# Autodesk Inventor assembly: 4x2
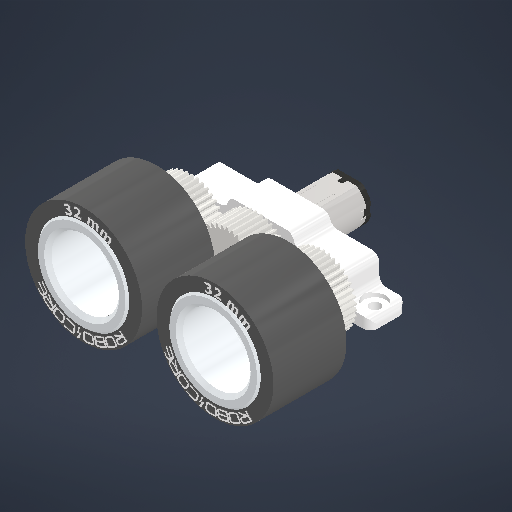
[picture p0: Inventor's stored thumbnail of the model, 512x512]
Saved by Autodesk Inventor 2026.1 (Build 301233020, 233B)
## iProperties
Created: 2026-02-10
Part Number: 4x2
Document SubType Name: Assembly
Designer: celio
Author: celio
## Documents named in this file (6)
- C:\Users\celio\OneDrive\Documentos\Inventor\ZeGuia\Montagem\4x2\Base\4x2.iam
- C:\Users\celio\OneDrive\Documentos\Inventor\ZeGuia\Roda\Roda.iam
- C:\Users\celio\OneDrive\Documentos\Inventor\ZeGuia\Motores\N20\N20 DC MOTOR.ipt
- C:\Users\celio\OneDrive\Documentos\Inventor\ZeGuia\Montagem\4x2\Suporte.ipt
- C:\Users\celio\OneDrive\Documentos\Inventor\ZeGuia\Montagem\4x2\Base\4x2\Design Accelerator\Engrenagens retas7.iam
- C:\Users\celio\OneDrive\Documentos\Inventor\ZeGuia\Montagem\4x2\Base\4x2\Design Accelerator\Engrenagens retas8.iam
## Components (7 placed, 4 different names)
1. Roda:1 [sub-assembly] — Tangente:1, Alinhado:3, Tangente:2, Tangente:4, Tangente:6, Rotação:4
2. Roda:2 [sub-assembly] — Tangente:1, Alinhado:2, Tangente:3, Tangente:5, Rotação:3
3. N20 DC MOTOR:1 — Coincidente:1, Coincidente:3, Alinhado:4, Coincidente:4, Alinhado:5, Rotativa:1
4. Suporte:1 — Alinhado:4, Coincidente:4, Alinhado:5, Inserir:1, Inserir:2
5. Engrenagens retas:1 [sub-assembly] — Inserir:1, Rotação:1, Rotação:3
6. Engrenagens retas:2 [sub-assembly] — Rotativa:1, Rotação:1, Rotação:2
7. Engrenagens retas:3 [sub-assembly] — Inserir:2, Rotação:2, Rotação:4
## Relationships (25: Tangent 6, Flush 4, RelateRotation 4, Angle 3, Mate 3, Symmetry 2, Insert 2, RevoluteJoint 1)
- Tangente:1 (4 mm): Roda:1 ↔ Roda:2
- Alinhado:2 [Flush] (-2 mm): Roda:2
- Alinhado:3 [Flush] (-2 mm): Roda:1
- Tangente:2: Roda:1
- Tangente:3: Roda:2
- Ângulo:1 [Angle] (0 deg)
- Tangente:4: Roda:1
- Simetria:1 [Symmetry]
- Coincidente:1 [Mate] (-5 mm): N20 DC MOTOR:1
- Ângulo:2 [Angle] (0 deg)
- Tangente:5: Roda:2
- Ângulo:3 [Angle] (0 deg)
- Tangente:6: Roda:1
- Simetria:2 [Symmetry]
- Coincidente:3 [Mate] (-6 mm): N20 DC MOTOR:1
- Alinhado:4 [Flush]: N20 DC MOTOR:1 ↔ Suporte:1
- Coincidente:4 [Mate]: N20 DC MOTOR:1 ↔ Suporte:1
- Alinhado:5 [Flush]: N20 DC MOTOR:1 ↔ Suporte:1
- Rotativa:1 [RevoluteJoint]: N20 DC MOTOR:1 ↔ Engrenagens retas:2
- Inserir:1 (1 mm): Suporte:1 ↔ Engrenagens retas:1
- Inserir:2 (1 mm): Suporte:1 ↔ Engrenagens retas:3
- Rotação:1 [RelateRotation] (1 ul): Engrenagens retas:1 ↔ Engrenagens retas:2
- Rotação:2 [RelateRotation] (1 ul): Engrenagens retas:2 ↔ Engrenagens retas:3
- Rotação:3 [RelateRotation] (1 ul): Roda:2 ↔ Engrenagens retas:1
- Rotação:4 [RelateRotation] (1 ul): Roda:1 ↔ Engrenagens retas:3
